# Autodesk Inventor assembly: ArmAssembly
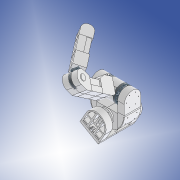
[picture p0: Inventor's stored thumbnail of the model, 180x180]
Saved by Autodesk Inventor 2017 SP1 (Build 210196100, 196)
## iProperties
Created: 2017-05-10
Part Number: ArmAssembly
Document SubType Name: Assembly
Designer: zallen
Author: zallen
## Documents named in this file (4)
- C:\Users\Zach\Documents\GitHub\cr-laundry-robot\src\Body\Arm Assembly\ArmAssembly.iam
- C:\Users\Zach\Documents\GitHub\cr-laundry-robot\src\Body\Arm Assembly\Shoulder Joint Assembly\Shoulder Joint Assembly.iam
- C:\Users\Zach\Documents\GitHub\cr-laundry-robot\src\Body\Arm Assembly\Bicep Assembly\BicepAssembly.iam
- C:\Users\Zach\Documents\GitHub\cr-laundry-robot\src\Body\Arm Assembly\Fore Arm Assembly\ForeArmAssembly.iam
## Components (3 placed, 3 different names)
1. Shoulder Joint Assembly:1 [sub-assembly] — Mate:67, Mate:68, Mate:69, Mate:70, Mate:71
2. BicepAssembly:1 [sub-assembly] — Mate:70, Mate:71, Mate:72, Mate:73
3. ForeArmAssembly:1 [sub-assembly] — Mate:72, Mate:73
## Relationships (7: Mate 7)
- Mate:67: Shoulder Joint Assembly:1
- Mate:68: Shoulder Joint Assembly:1
- Mate:69: Shoulder Joint Assembly:1
- Mate:70: Shoulder Joint Assembly:1 ↔ BicepAssembly:1
- Mate:71: Shoulder Joint Assembly:1 ↔ BicepAssembly:1
- Mate:72: BicepAssembly:1 ↔ ForeArmAssembly:1
- Mate:73: BicepAssembly:1 ↔ ForeArmAssembly:1
